# Autodesk Inventor assembly: Chain Drive
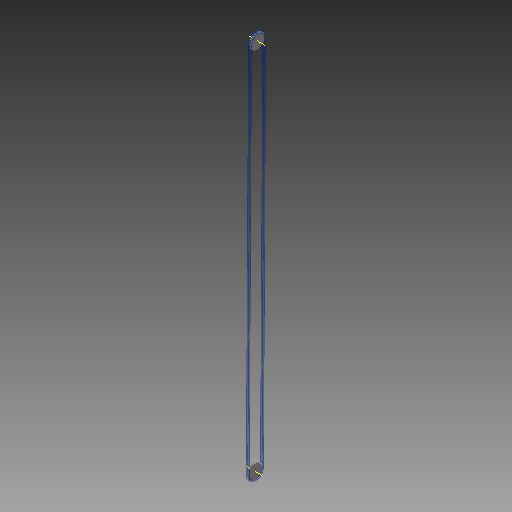
[picture p0: Inventor's stored thumbnail of the model, 512x512]
Saved by Autodesk Inventor 2017 (Build 210142000, 142)
## iProperties
ClientObjectVersion: 1
Created: 2017-12-29
Part Number: Chain Drive
Document SubType Name: Assembly
Designer: Micah
Author: Micah
## Documents named in this file (4)
- C:\Users\Micah\Desktop\inventor\CADathon-2017\2AM-17-A-0200 - Smokestack Elevator\2AM-17-A-0200 - elevator\Design Accelerator\Chain Drive7.iam
- C:\Users\Micah\Desktop\inventor\CADathon-2017\2AM-17-A-0200 - Smokestack Elevator\2AM-17-A-0200 - elevator\Design Accelerator\Roller Chain7.ipt
- C:\Users\Micah\Desktop\inventor\CADathon-2017\2AM-17-A-0200 - Smokestack Elevator\2AM-17-A-0200 - elevator\Design Accelerator\Roller Chain Sprocket17.ipt
- C:\Users\Micah\Desktop\inventor\CADathon-2017\2AM-17-A-0200 - Smokestack Elevator\2AM-17-A-0200 - elevator\Design Accelerator\Roller Chain Sprocket27.ipt
## Components (3 placed, 3 different names)
1. Roller Chain:1 — Flush:1, Mate:1, Mate:2, Flush:2, Mate:3, Mate:4
2. Roller Chain Sprocket1:1 — Flush:1, Mate:1, Mate:2, Rotation:1
3. Roller Chain Sprocket2:1 — Flush:2, Mate:3, Rotation:1, Mate:4
## Relationships (7: Mate 4, Flush 2, RelateRotation 1)
- Flush:1: Roller Chain:1 ↔ Roller Chain Sprocket1:1
- Mate:1: Roller Chain:1 ↔ Roller Chain Sprocket1:1
- Mate:2: Roller Chain:1 ↔ Roller Chain Sprocket1:1
- Flush:2: Roller Chain:1 ↔ Roller Chain Sprocket2:1
- Mate:3: Roller Chain:1 ↔ Roller Chain Sprocket2:1
- Rotation:1 [RelateRotation] (1 ul): Roller Chain Sprocket1:1 ↔ Roller Chain Sprocket2:1
- Mate:4: Roller Chain:1 ↔ Roller Chain Sprocket2:1
